# Autodesk Inventor assembly: Gestikulaser
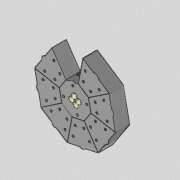
[picture p0: Inventor's stored thumbnail of the model, 180x180]
Saved by Autodesk Inventor 2018.2 (Build 222227000, 227)
## iProperties
Created: 2018-11-01
Part Number: Gestikulaser
Material: Generisch
Document SubType Name: Assembly
Designer: M.Knabel
Author: M.Knabel
## Documents named in this file (3)
- V:\A340\2018\DOKUMENTATION\COSIMA\COSIMA-Laserstar\CAD\Gestikulaser.iam
- V:\A340\2018\DOKUMENTATION\COSIMA\COSIMA-Laserstar\CAD\Oktokommander\Oktokommander.iam
- V:\A340\2018\DOKUMENTATION\COSIMA\COSIMA-Laserstar\CAD\Detektormodul\Detektormodul.iam
## Components (8 placed, 2 different names)
1. Oktokommander:1 [sub-assembly] — Passend:1, Passend:2, Passend:3, Fluchtend:1, Passend:4, Fluchtend:2, Fluchtend:3, Passend:5, Fluchtend:4, Fluchtend:5, Fluchtend:6, Fluchtend:7, Fluchtend:8, Fluchtend:10, Passend:14, Passend:15, Passend:16, Passend:17, Passend:18, Fluchtend:11, Fluchtend:12, Fluchtend:13, Fluchtend:14, Fluchtend:15, Passend:19, Passend:20, Passend:21
2. Detektormodul:1 [sub-assembly] — Fluchtend:1, Passend:4, Fluchtend:2
3. Detektormodul:2 [sub-assembly] — Fluchtend:3, Passend:5, Fluchtend:4
4. Detektormodul:3 [sub-assembly] — Fluchtend:10, Passend:14, Fluchtend:15
5. Detektormodul:5 [sub-assembly] — Fluchtend:8, Passend:18, Fluchtend:11, Passend:21
6. Detektormodul:6 [sub-assembly] — Fluchtend:7, Passend:17, Fluchtend:12, Passend:20
7. Detektormodul:7 [sub-assembly] — Fluchtend:5, Passend:16, Fluchtend:13, Passend:19
8. Detektormodul:8 [sub-assembly] — Fluchtend:6, Passend:15, Fluchtend:14
## Relationships (27: Flush 14, Mate 13)
- Passend:1 [Mate]: Oktokommander:1
- Passend:2 [Mate]: Oktokommander:1
- Passend:3 [Mate]: Oktokommander:1
- Fluchtend:1 [Flush]: Oktokommander:1 ↔ Detektormodul:1
- Passend:4 [Mate]: Oktokommander:1 ↔ Detektormodul:1
- Fluchtend:2 [Flush]: Oktokommander:1 ↔ Detektormodul:1
- Fluchtend:3 [Flush]: Oktokommander:1 ↔ Detektormodul:2
- Passend:5 [Mate]: Oktokommander:1 ↔ Detektormodul:2
- Fluchtend:4 [Flush]: Oktokommander:1 ↔ Detektormodul:2
- Fluchtend:5 [Flush]: Oktokommander:1 ↔ Detektormodul:7
- Fluchtend:6 [Flush]: Oktokommander:1 ↔ Detektormodul:8
- Fluchtend:7 [Flush]: Oktokommander:1 ↔ Detektormodul:6
- Fluchtend:8 [Flush]: Oktokommander:1 ↔ Detektormodul:5
- Fluchtend:10 [Flush]: Oktokommander:1 ↔ Detektormodul:3
- Passend:14 [Mate]: Oktokommander:1 ↔ Detektormodul:3
- Passend:15 [Mate]: Oktokommander:1 ↔ Detektormodul:8
- Passend:16 [Mate]: Oktokommander:1 ↔ Detektormodul:7
- Passend:17 [Mate]: Oktokommander:1 ↔ Detektormodul:6
- Passend:18 [Mate]: Oktokommander:1 ↔ Detektormodul:5
- Fluchtend:11 [Flush]: Oktokommander:1 ↔ Detektormodul:5
- Fluchtend:12 [Flush]: Oktokommander:1 ↔ Detektormodul:6
- Fluchtend:13 [Flush]: Oktokommander:1 ↔ Detektormodul:7
- Fluchtend:14 [Flush]: Oktokommander:1 ↔ Detektormodul:8
- Fluchtend:15 [Flush]: Oktokommander:1 ↔ Detektormodul:3
- Passend:19 [Mate] (50 mm): Oktokommander:1 ↔ Detektormodul:7
- Passend:20 [Mate] (50 mm): Oktokommander:1 ↔ Detektormodul:6
- Passend:21 [Mate] (50 mm): Oktokommander:1 ↔ Detektormodul:5
